# Autodesk Inventor assembly: mech_assembly-right_b
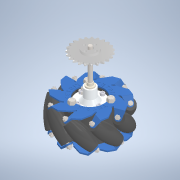
[picture p0: Inventor's stored thumbnail of the model, 180x180]
Saved by Autodesk Inventor 2020 (Build 240168000, 168)
## iProperties
Created: 2019-09-11
Part Number: mech_assembly-right_b
Document SubType Name: Assembly
Designer: tbloo
Author: tbloo
## Documents named in this file (6)
- D:\Documents\GitHub\AO_Robotics\CAD\Projects\Timothy Bloot\mech_assembly-right_b.iam
- D:\Documents\GitHub\AO_Robotics\CAD\Parts Kits\FTC Tetrix KOP Organized (7-24-19)\Axle Hardware\Tetrix_40225-80mm.ipt
- D:\Documents\GitHub\AO_Robotics\CAD\Parts Kits\FTC Tetrix KOP Organized (7-24-19)\Axle Hardware\AM_6mm_Bushing.ipt
- D:\Documents\GitHub\AO_Robotics\CAD\Parts Kits\FTC Tetrix KOP Organized (7-24-19)\Axle Hardware\Tetrix_39079.iam
- D:\Documents\GitHub\AO_Robotics\CAD\Parts Kits\FTC Tetrix KOP Organized (7-24-19)\Gear\Tetrix_39169.ipt
- D:\Documents\GitHub\AO_Robotics\CAD\Parts Kits\FTC Tetrix KOP Organized (7-24-19)\Wheel\Mechanum Wheel\right_b_mecanum wheel.ipt
## Components (6 placed, 5 different names)
1. Tetrix_40225-80mm:1 — Rotational:3, Rigid:1, Rigid:3
2. AM_6mm_Bushing:2 — Rotational:3
3. Tetrix_39079:1 [sub-assembly] — Rigid:1, Rigid:2
4. Tetrix_39169:1 — Rigid:2
5. right_b_mecanum wheel:1 — Rigid:3, Rotational:4
6. AM_6mm_Bushing:3 — Rotational:4
## Relationships (5: WeldJoint 3, RevoluteJoint 2)
- Rotational:3 [RevoluteJoint] (-18.3 mm): Tetrix_40225-80mm:1 ↔ AM_6mm_Bushing:2
- Rigid:1 [WeldJoint] (-16.3 mm): Tetrix_40225-80mm:1 ↔ Tetrix_39079:1
- Rigid:2 [WeldJoint]: Tetrix_39079:1 ↔ Tetrix_39169:1
- Rigid:3 [WeldJoint]: Tetrix_40225-80mm:1 ↔ right_b_mecanum wheel:1
- Rotational:4 [RevoluteJoint]: right_b_mecanum wheel:1 ↔ AM_6mm_Bushing:3
